# Autodesk Inventor assembly: FM1410P
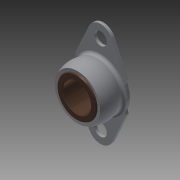
[picture p0: Inventor's stored thumbnail of the model, 180x180]
Saved by Autodesk Inventor 2013 (Build 170138000, 138)
## iProperties
Category: Miscellaneous
Company: Autodesk Inc.
Created: 2012-12-03
Part Number: FM1410P
Document SubType Name: Assembly
Designer: Autodesk Inc.
Catalog Web Link: http://www.triangleoshkosh.com/eng/products/self-aligning-sleeve-bearings/flange-mounted-bearings/side-flange-mounted-bearings-miniature
Description: Flange mount 5/8" bronze bearing
Vendor: Triangle Manufacturing
Author: Autodesk Inc.
## Documents named in this file (3)
- C:\Data Folder\FIRST 2013\FIRST KOP\Parts\Miscellaneous\MISC_SideFlangeBearings_FM1410.iam
- C:\Data Folder\FIRST 2013\FIRST KOP\Parts\Miscellaneous\MISC_FlangeMount_4050.ipt
- C:\Data Folder\FIRST 2013\FIRST KOP\Parts\Miscellaneous\Misc_BearingBall_Triangle_1410P.ipt
## Components (2 placed, 2 different names)
1. MISC_FlangeMount_4050:1 — Mate:1, Tangent:1
2. Misc_BearingBall_Triangle_1410P:1 — Mate:1, Tangent:1
## Relationships (2: Mate 1, Tangent 1)
- Mate:1: MISC_FlangeMount_4050:1 ↔ Misc_BearingBall_Triangle_1410P:1
- Tangent:1: MISC_FlangeMount_4050:1 ↔ Misc_BearingBall_Triangle_1410P:1
